# Autodesk Inventor assembly: AssemblySpring
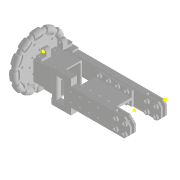
[picture p0: Inventor's stored thumbnail of the model, 180x180]
Saved by Autodesk Inventor 2022 (Build 260153000, 153)
## iProperties
Created: 2022-11-21
Part Number: AssemblySpring
Document SubType Name: Assembly
Designer: MVeszpremi
Author: MVeszpremi
## Documents named in this file (7)
- C:\Users\veszp\Dropbox\180DAB CAD\SpringLoadedDesign\AssemblySpring.iam
- C:\Users\veszp\Dropbox\180DAB CAD\SpringLoadedDesign\StepperMotorHolder_Spring.ipt
- C:\Users\veszp\Dropbox\180DAB CAD\SpringLoadedDesign\RobotBaseMotorExtUpper_Spring.ipt
- C:\Users\veszp\Dropbox\180DAB CAD\SpringLoadedDesign\RobotBaseMotorExtLower_Spring.ipt
- C:\Users\veszp\Dropbox\180DAB CAD\SpringLoadedDesign\SpringConn.ipt
- C:\Users\veszp\Dropbox\180DAB CAD\SpringLoadedDesign\ExtConnector_Spring.ipt
- C:\Users\veszp\Dropbox\180DAB CAD\Wheel.ipt
## Components (7 placed, 6 different names)
1. StepperMotorHolder_Spring:1 — Mate:2, Mate:3, Mate:9, Mate:10, Mate:16, Mate:17
2. RobotBaseMotorExtUpper_Spring:1 — Mate:2, Mate:3, Mate:4, Mate:5, Mate:6, Mate:13, Mate:14
3. RobotBaseMotorExtLower_Spring:1 — Mate:4, Mate:5, Mate:6, Mate:7, Mate:8, Mate:12, Mate:15
4. SpringConn:1 — Mate:7, Mate:8, Angle:1, Mate:11
5. SpringConn:2 — Mate:9, Mate:10, Angle:1, Mate:11
6. ExtConnector_Spring:1 — Mate:12, Mate:13, Mate:14, Mate:15
7. Wheel:1 — Mate:16, Mate:17
## Relationships (17: Mate 16, Angle 1)
- Mate:2 (0.5 mm): StepperMotorHolder_Spring:1 ↔ RobotBaseMotorExtUpper_Spring:1
- Mate:3: StepperMotorHolder_Spring:1 ↔ RobotBaseMotorExtUpper_Spring:1
- Mate:4: RobotBaseMotorExtUpper_Spring:1 ↔ RobotBaseMotorExtLower_Spring:1
- Mate:5: RobotBaseMotorExtUpper_Spring:1 ↔ RobotBaseMotorExtLower_Spring:1
- Mate:6 (55 mm): RobotBaseMotorExtUpper_Spring:1 ↔ RobotBaseMotorExtLower_Spring:1
- Mate:7: RobotBaseMotorExtLower_Spring:1 ↔ SpringConn:1
- Mate:8: RobotBaseMotorExtLower_Spring:1 ↔ SpringConn:1
- Mate:9: StepperMotorHolder_Spring:1 ↔ SpringConn:2
- Mate:10: StepperMotorHolder_Spring:1 ↔ SpringConn:2
- Angle:1 (180 deg): SpringConn:1 ↔ SpringConn:2
- Mate:11: SpringConn:1 ↔ SpringConn:2
- Mate:12: RobotBaseMotorExtLower_Spring:1 ↔ ExtConnector_Spring:1
- Mate:13: RobotBaseMotorExtUpper_Spring:1 ↔ ExtConnector_Spring:1
- Mate:14: RobotBaseMotorExtUpper_Spring:1 ↔ ExtConnector_Spring:1
- Mate:15: RobotBaseMotorExtLower_Spring:1 ↔ ExtConnector_Spring:1
- Mate:16: StepperMotorHolder_Spring:1 ↔ Wheel:1
- Mate:17 (10 mm): StepperMotorHolder_Spring:1 ↔ Wheel:1
